# Autodesk Inventor assembly: SC700-40kg_Cover
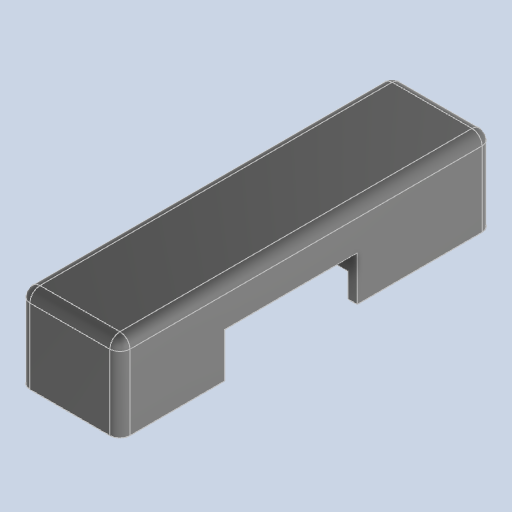
[picture p0: Inventor's stored thumbnail of the model, 512x512]
Saved by Autodesk Inventor 2022.5 (Build 265521000, 521)
## iProperties
Created: 2023-05-14
Part Number: SC700-40kg_Cover
Document SubType Name: Assembly
Designer: Masato Kubotera
Author: Masato Kubotera
## Documents named in this file (3)
- C:\Users\Masato\Documents\Inventor\SUSTAINA-OP\ModelingFiles\LowerBody\Foot\SC700-40kg_Cover.iam
- C:\Users\Masato\Documents\Inventor\SUSTAINA-OP\ModelingFiles\LowerBody\Foot\SC700-40kg_Cover.ipt
- C:\Users\Masato\Documents\Inventor\SUSTAINA-OP\ModelingFiles\COTS\InsertNut\UD-43040.ipt
## Components (3 placed, 2 different names)
1. SC700-40kg_Cover:1 — フラッシュ:1, フラッシュ:2, フラッシュ:3, 挿入:1, 挿入:2
2. UD-43040:1 — 挿入:1
3. UD-43040:2 — 挿入:2
## Relationships (5: Flush 3, Insert 2)
- フラッシュ:1 [Flush]: SC700-40kg_Cover:1
- フラッシュ:2 [Flush]: SC700-40kg_Cover:1
- フラッシュ:3 [Flush]: SC700-40kg_Cover:1
- 挿入:1 [Insert]: SC700-40kg_Cover:1 ↔ UD-43040:1
- 挿入:2 [Insert]: SC700-40kg_Cover:1 ↔ UD-43040:2
